# Autodesk Inventor assembly: scintillatorPanel
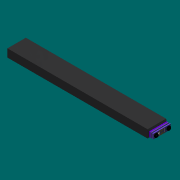
[picture p0: Inventor's stored thumbnail of the model, 180x180]
Saved by Autodesk Inventor 2016 SP1 (Build 200210100, 210)
## iProperties
Created: 2016-02-15
Part Number: scintillatorPanel
Document SubType Name: Assembly
Designer: sawai
Author: sawai
## Documents named in this file (5)
- C:\Users\sawai\OneDrive\projects\scintillatorPanel\scintillatorPanel.iam
- C:\Users\sawai\OneDrive\projects\scintillatorPanel\panel.iam
- C:\Users\sawai\OneDrive\projects\scintillatorPanel\mppcSensorInterface\cad\sensorBoard.iam
- C:\Users\sawai\OneDrive\projects\scintillatorPanel\edgeCoating.ipt
- C:\Users\sawai\OneDrive\projects\scintillatorPanel\4-40x0.5in.ipt
## Components (5 placed, 4 different names)
1. panel:1 [sub-assembly] — Mate:1, Angle:1, Mate:2, Flush:1
2. sensorBoard:1 [sub-assembly] — Mate:1, Angle:1, Mate:2, Mate:3, Mate:4, Mate:5, Mate:6
3. edgeCoating:1 — Flush:1
4. 4-40x0.5in:1 — Mate:3, Mate:5
5. 4-40x0.5in:2 — Mate:4, Mate:6
## Relationships (8: Mate 6, Angle 1, Flush 1)
- Mate:1: panel:1 ↔ sensorBoard:1
- Angle:1 (0 deg): panel:1 ↔ sensorBoard:1
- Mate:2: panel:1 ↔ sensorBoard:1
- Flush:1: panel:1 ↔ edgeCoating:1
- Mate:3: sensorBoard:1 ↔ 4-40x0.5in:1
- Mate:4: sensorBoard:1 ↔ 4-40x0.5in:2
- Mate:5: sensorBoard:1 ↔ 4-40x0.5in:1
- Mate:6: sensorBoard:1 ↔ 4-40x0.5in:2
